# Autodesk Inventor assembly: AK-C-C10-Wallsl
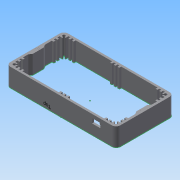
[picture p0: Inventor's stored thumbnail of the model, 180x180]
Saved by Autodesk Inventor 2016 (Build 200138000, 138)
## iProperties
Created: 2016-03-30
Part Number: AK-C-C10-Wallsl
Document SubType Name: Assembly
Designer: admin
Author: admin
## Documents named in this file (3)
- E:\Alex\HS-Spectrophotometer\parts\New vesion\SZOMK-AK-C-C10-Walls.iam
- E:\Alex\HS-Spectrophotometer\parts\New vesion\AK-C-C10-Left_wall.ipt
- E:\Alex\HS-Spectrophotometer\parts\New vesion\AK-C-C10-Right_wall.ipt
## Components (2 placed, 2 different names)
1. AK-C-C10-Left_wall:1 — Mate:1, Flush:1, Flush:2
2. AK-C-C10-Right_wall:1 — Mate:1, Flush:1, Flush:2
## Relationships (3: Flush 2, Mate 1)
- Mate:1: AK-C-C10-Left_wall:1 ↔ AK-C-C10-Right_wall:1
- Flush:1: AK-C-C10-Left_wall:1 ↔ AK-C-C10-Right_wall:1
- Flush:2: AK-C-C10-Left_wall:1 ↔ AK-C-C10-Right_wall:1
